# Autodesk Inventor assembly: ODrive S1 Housing Assembly
(part 2 of 2)
- C:\Users\seene\OneDrive\SBRT\Robocup Rescue\Chassis\Electronics Box\ODrive S1 Housing Assembly\C_0805_2012Metric_3.ipt
- C:\Users\seene\OneDrive\SBRT\Robocup Rescue\Chassis\Electronics Box\ODrive S1 Housing Assembly\_X2_8010632F54C130B130FC30B903A6_X0_10x9.5L_SIDE_CODE_G_3.ipt
- C:\Users\seene\OneDrive\SBRT\Robocup Rescue\Chassis\Electronics Box\ODrive S1 Housing Assembly\ASMPH-0806.ipt
- C:\Users\seene\OneDrive\SBRT\Robocup Rescue\Chassis\Electronics Box\ODrive S1 Housing Assembly\Extruded_1_1.ipt
- C:\Users\seene\OneDrive\SBRT\Robocup Rescue\Chassis\Electronics Box\ODrive S1 Housing Assembly\R_0402_1005Metric_65.ipt
- C:\Users\seene\OneDrive\SBRT\Robocup Rescue\Chassis\Electronics Box\ODrive S1 Housing Assembly\SOP_Advance(N)_(1)_11.ipt
- C:\Users\seene\OneDrive\SBRT\Robocup Rescue\Chassis\Electronics Box\ODrive S1 Housing Assembly\SOP_Advance(N)_(1)_2_4.ipt
- C:\Users\seene\OneDrive\SBRT\Robocup Rescue\Chassis\Electronics Box\ODrive S1 Housing Assembly\SOP_Advance(N)_(1)_5_4.ipt
- C:\Users\seene\OneDrive\SBRT\Robocup Rescue\Chassis\Electronics Box\ODrive S1 Housing Assembly\Open_CASCADE_STEP_translator_6.8_48.4.1_30.ipt
- C:\Users\seene\OneDrive\SBRT\Robocup Rescue\Chassis\Electronics Box\ODrive S1 Housing Assembly\Open_CASCADE_STEP_translator_6.8_48.4.1_26.ipt
- C:\Users\seene\OneDrive\SBRT\Robocup Rescue\Chassis\Electronics Box\ODrive S1 Housing Assembly\Open_CASCADE_STEP_translator_6.8_48.4.1_46.ipt
- C:\Users\seene\OneDrive\SBRT\Robocup Rescue\Chassis\Electronics Box\ODrive S1 Housing Assembly\Open_CASCADE_STEP_translator_6.8_48.4.1_42.ipt
- C:\Users\seene\OneDrive\SBRT\Robocup Rescue\Chassis\Electronics Box\ODrive S1 Housing Assembly\Open_CASCADE_STEP_translator_6.8_48.4.1_62.ipt
- C:\Users\seene\OneDrive\SBRT\Robocup Rescue\Chassis\Electronics Box\ODrive S1 Housing Assembly\Open_CASCADE_STEP_translator_6.8_48.4.1_58.ipt
- C:\Users\seene\OneDrive\SBRT\Robocup Rescue\Chassis\Electronics Box\ODrive S1 Housing Assembly\R_0402_1005Metric_25.ipt
- C:\Users\seene\OneDrive\SBRT\Robocup Rescue\Chassis\Electronics Box\ODrive S1 Housing Assembly\R_0402_1005Metric_21.ipt
- C:\Users\seene\OneDrive\SBRT\Robocup Rescue\Chassis\Electronics Box\ODrive S1 Housing Assembly\Open_CASCADE_STEP_translator_6.8_48.2.1.ipt
- C:\Users\seene\OneDrive\SBRT\Robocup Rescue\Chassis\Electronics Box\ODrive S1 Housing Assembly\Open_CASCADE_STEP_translator_6.8_56.4.1_5.ipt
- C:\Users\seene\OneDrive\SBRT\Robocup Rescue\Chassis\Electronics Box\ODrive S1 Housing Assembly\Leader_3_1.ipt
- C:\Users\seene\OneDrive\SBRT\Robocup Rescue\Chassis\Electronics Box\ODrive S1 Housing Assembly\Open_CASCADE_STEP_translator_6.8_5.2.1.ipt
- C:\Users\seene\OneDrive\SBRT\Robocup Rescue\Chassis\Electronics Box\ODrive S1 Housing Assembly\Open_CASCADE_STEP_translator_6.8_48.2.1_1.ipt
- C:\Users\seene\OneDrive\SBRT\Robocup Rescue\Chassis\Electronics Box\ODrive S1 Housing Assembly\Leader_15.ipt
- C:\Users\seene\OneDrive\SBRT\Robocup Rescue\Chassis\Electronics Box\ODrive S1 Housing Assembly\Open_CASCADE_STEP_translator_6.8_48.4.1_14.ipt
- C:\Users\seene\OneDrive\SBRT\Robocup Rescue\Chassis\Electronics Box\ODrive S1 Housing Assembly\Open_CASCADE_STEP_translator_6.8_48.4.1_10.ipt
- C:\Users\seene\OneDrive\SBRT\Robocup Rescue\Chassis\Electronics Box\ODrive S1 Housing Assembly\R_0402_1005Metric_13.ipt
- C:\Users\seene\OneDrive\SBRT\Robocup Rescue\Chassis\Electronics Box\ODrive S1 Housing Assembly\_X2_8010632F54C15EA77248752888DC52A97AEF5B5003A6_X0_10_SIZE_CODE_G_1.ipt
- C:\Users\seene\OneDrive\SBRT\Robocup Rescue\Chassis\Electronics Box\ODrive S1 Housing Assembly\C_0402_1005Metric_10.ipt
- C:\Users\seene\OneDrive\SBRT\Robocup Rescue\Chassis\Electronics Box\ODrive S1 Housing Assembly\Open_CASCADE_STEP_translator_6.8_34.4.1_7.ipt
- C:\Users\seene\OneDrive\SBRT\Robocup Rescue\Chassis\Electronics Box\ODrive S1 Housing Assembly\Open_CASCADE_STEP_translator_6.8_34.4.1_3.ipt
- C:\Users\seene\OneDrive\SBRT\Robocup Rescue\Chassis\Electronics Box\ODrive S1 Housing Assembly\Open_CASCADE_STEP_translator_6.8_41.4.1_4.ipt
- C:\Users\seene\OneDrive\SBRT\Robocup Rescue\Chassis\Electronics Box\ODrive S1 Housing Assembly\Open_CASCADE_STEP_translator_6.8_41.4.1.ipt
- C:\Users\seene\OneDrive\SBRT\Robocup Rescue\Chassis\Electronics Box\ODrive S1 Housing Assembly\Cylinder_4_1.ipt
- C:\Users\seene\OneDrive\SBRT\Robocup Rescue\Chassis\Electronics Box\ODrive S1 Housing Assembly\B0-6.3-0-2512_1.ipt
- C:\Users\seene\OneDrive\SBRT\Robocup Rescue\Chassis\Electronics Box\ODrive S1 Housing Assembly\Cylinder_17.ipt
- C:\Users\seene\OneDrive\SBRT\Robocup Rescue\Chassis\Electronics Box\ODrive S1 Housing Assembly\Cylinder_13.ipt
- C:\Users\seene\OneDrive\SBRT\Robocup Rescue\Chassis\Electronics Box\ODrive S1 Housing Assembly\Cylinder_7_1.ipt
- C:\Users\seene\OneDrive\SBRT\Robocup Rescue\Chassis\Electronics Box\ODrive S1 Housing Assembly\C_0603_1608Metric_9.ipt
- C:\Users\seene\OneDrive\SBRT\Robocup Rescue\Chassis\Electronics Box\ODrive S1 Housing Assembly\C_0603_1608Metric_5.ipt
- C:\Users\seene\OneDrive\SBRT\Robocup Rescue\Chassis\Electronics Box\ODrive S1 Housing Assembly\Pins_7.ipt
- C:\Users\seene\OneDrive\SBRT\Robocup Rescue\Chassis\Electronics Box\ODrive S1 Housing Assembly\C_0603_1608Metric.ipt
- C:\Users\seene\OneDrive\SBRT\Robocup Rescue\Chassis\Electronics Box\ODrive S1 Housing Assembly\lead_2.ipt
- C:\Users\seene\OneDrive\SBRT\Robocup Rescue\Chassis\Electronics Box\ODrive S1 Housing Assembly\Open_CASCADE_STEP_translator_6.8_2.3.1_11.ipt
- C:\Users\seene\OneDrive\SBRT\Robocup Rescue\Chassis\Electronics Box\ODrive S1 Housing Assembly\Open_CASCADE_STEP_translator_6.8_2.2.1_1.ipt
- C:\Users\seene\OneDrive\SBRT\Robocup Rescue\Chassis\Electronics Box\ODrive S1 Housing Assembly\_Dual_s.ipt
- C:\Users\seene\OneDrive\SBRT\Robocup Rescue\Chassis\Electronics Box\ODrive S1 Housing Assembly\R_0402_1005Metric_32.ipt
- C:\Users\seene\OneDrive\SBRT\Robocup Rescue\Chassis\Electronics Box\ODrive S1 Housing Assembly\R_0402_1005Metric_46.ipt
- C:\Users\seene\OneDrive\SBRT\Robocup Rescue\Chassis\Electronics Box\ODrive S1 Housing Assembly\HCS2512_L500_stp_1_2.ipt
- C:\Users\seene\OneDrive\SBRT\Robocup Rescue\Chassis\Electronics Box\ODrive S1 Housing Assembly\Open_CASCADE_STEP_translator_6.8_48.4.1_5.ipt
- C:\Users\seene\OneDrive\SBRT\Robocup Rescue\Chassis\Electronics Box\ODrive S1 Housing Assembly\Open_CASCADE_STEP_translator_6.8_48.4.1_21.ipt
- C:\Users\seene\OneDrive\SBRT\Robocup Rescue\Chassis\Electronics Box\ODrive S1 Housing Assembly\Open_CASCADE_STEP_translator_6.8_48.4.1_37.ipt
- C:\Users\seene\OneDrive\SBRT\Robocup Rescue\Chassis\Electronics Box\ODrive S1 Housing Assembly\Open_CASCADE_STEP_translator_6.8_48.4.1_53.ipt
- C:\Users\seene\OneDrive\SBRT\Robocup Rescue\Chassis\Electronics Box\ODrive S1 Housing Assembly\Leader_4_2.ipt
- C:\Users\seene\OneDrive\SBRT\Robocup Rescue\Chassis\Electronics Box\ODrive S1 Housing Assembly\Open_CASCADE_STEP_translator_6.8_56.4.1.ipt
- C:\Users\seene\OneDrive\SBRT\Robocup Rescue\Chassis\Electronics Box\ODrive S1 Housing Assembly\Leader_6_1.ipt
- C:\Users\seene\OneDrive\SBRT\Robocup Rescue\Chassis\Electronics Box\ODrive S1 Housing Assembly\Leader_10.ipt
- C:\Users\seene\OneDrive\SBRT\Robocup Rescue\Chassis\Electronics Box\ODrive S1 Housing Assembly\C_0402_1005Metric_31.ipt
- C:\Users\seene\OneDrive\SBRT\Robocup Rescue\Chassis\Electronics Box\ODrive S1 Housing Assembly\C_0805_1MM_2_1.ipt
- C:\Users\seene\OneDrive\SBRT\Robocup Rescue\Chassis\Electronics Box\ODrive S1 Housing Assembly\C_0805_1MM.ipt
- C:\Users\seene\OneDrive\SBRT\Robocup Rescue\Chassis\Electronics Box\ODrive S1 Housing Assembly\_X2_8010632F54C130EA30FC30C97DDA03A6_X0_10_SIZE_CODE_G_3.ipt
- C:\Users\seene\OneDrive\SBRT\Robocup Rescue\Chassis\Electronics Box\ODrive S1 Housing Assembly\_X2_8010632F54C15EA7724803A6_X0_10_SIZE_CODE_G_1.ipt
- C:\Users\seene\OneDrive\SBRT\Robocup Rescue\Chassis\Electronics Box\ODrive S1 Housing Assembly\R_0402_1005Metric_11.ipt
- C:\Users\seene\OneDrive\SBRT\Robocup Rescue\Chassis\Electronics Box\ODrive S1 Housing Assembly\C_0603_1608Metric_28.ipt
- C:\Users\seene\OneDrive\SBRT\Robocup Rescue\Chassis\Electronics Box\ODrive S1 Housing Assembly\_X2_8010632F54C130EA30FC30C97DDA03A6_X0_10_SIZE_CODE_G_7.ipt
- C:\Users\seene\OneDrive\SBRT\Robocup Rescue\Chassis\Electronics Box\ODrive S1 Housing Assembly\B0-6.3-0-2512_3.ipt
- C:\Users\seene\OneDrive\SBRT\Robocup Rescue\Chassis\Electronics Box\ODrive S1 Housing Assembly\C_0603_1608Metric_33.ipt
- C:\Users\seene\OneDrive\SBRT\Robocup Rescue\Chassis\Electronics Box\ODrive S1 Housing Assembly\C_0603_1608Metric_31.ipt
- C:\Users\seene\OneDrive\SBRT\Robocup Rescue\Chassis\Electronics Box\ODrive S1 Housing Assembly\Open_CASCADE_STEP_translator_6.8_34.2.1.ipt
- C:\Users\seene\OneDrive\SBRT\Robocup Rescue\Chassis\Electronics Box\ODrive S1 Housing Assembly\SOP_Advance(N)_(1)_6_3.ipt
- C:\Users\seene\OneDrive\SBRT\Robocup Rescue\Chassis\Electronics Box\ODrive S1 Housing Assembly\Open_CASCADE_STEP_translator_6.8_2.3.1_4.ipt
- C:\Users\seene\OneDrive\SBRT\Robocup Rescue\Chassis\Electronics Box\ODrive S1 Housing Assembly\_X2_00C700D000B300FD_X0_-_X2_00C000AD00C900EC_X0_2.ipt
- C:\Users\seene\OneDrive\SBRT\Robocup Rescue\Chassis\Electronics Box\ODrive S1 Housing Assembly\C_0603_1608Metric_1.ipt
- C:\Users\seene\OneDrive\SBRT\Robocup Rescue\Chassis\Electronics Box\ODrive S1 Housing Assembly\C_0402_1005Metric_13.ipt
- C:\Users\seene\OneDrive\SBRT\Robocup Rescue\Chassis\Electronics Box\ODrive S1 Housing Assembly\D_SOD-123F_5.ipt
- C:\Users\seene\OneDrive\SBRT\Robocup Rescue\Chassis\Electronics Box\ODrive S1 Housing Assembly\Cylinder_11.ipt
- C:\Users\seene\OneDrive\SBRT\Robocup Rescue\Chassis\Electronics Box\ODrive S1 Housing Assembly\M3Ò»×ÖÆ½Ô²Í·ÂÝ¶¤.ipt
- C:\Users\seene\OneDrive\SBRT\Robocup Rescue\Chassis\Electronics Box\ODrive S1 Housing Assembly\C_0402_1005Metric_23.ipt
- C:\Users\seene\OneDrive\SBRT\Robocup Rescue\Chassis\Electronics Box\ODrive S1 Housing Assembly\C_0402_1005Metric_19.ipt
- C:\Users\seene\OneDrive\SBRT\Robocup Rescue\Chassis\Electronics Box\ODrive S1 Housing Assembly\Cylinder_24.ipt
- C:\Users\seene\OneDrive\SBRT\Robocup Rescue\Chassis\Electronics Box\ODrive S1 Housing Assembly\R_0402_1005Metric_5.ipt
- C:\Users\seene\OneDrive\SBRT\Robocup Rescue\Chassis\Electronics Box\ODrive S1 Housing Assembly\SOP_Advance(N)_(1)_1_4.ipt
- C:\Users\seene\OneDrive\SBRT\Robocup Rescue\Chassis\Electronics Box\ODrive S1 Housing Assembly\SOP_Advance(N)_(1)_12.ipt
- C:\Users\seene\OneDrive\SBRT\Robocup Rescue\Chassis\Electronics Box\ODrive S1 Housing Assembly\SOP_Advance(N)_(1)_4_4.ipt
- C:\Users\seene\OneDrive\SBRT\Robocup Rescue\Chassis\Electronics Box\ODrive S1 Housing Assembly\SOP_Advance(N)_(1)_3_5.ipt
- C:\Users\seene\OneDrive\SBRT\Robocup Rescue\Chassis\Electronics Box\ODrive S1 Housing Assembly\SOP_Advance(N)_(1)_6_4.ipt
- C:\Users\seene\OneDrive\SBRT\Robocup Rescue\Chassis\Electronics Box\ODrive S1 Housing Assembly\R_0402_1005Metric_41.ipt
- C:\Users\seene\OneDrive\SBRT\Robocup Rescue\Chassis\Electronics Box\ODrive S1 Housing Assembly\R_0402_1005Metric_37.ipt
- C:\Users\seene\OneDrive\SBRT\Robocup Rescue\Chassis\Electronics Box\ODrive S1 Housing Assembly\R_0603_1608Metric_2.ipt
- C:\Users\seene\OneDrive\SBRT\Robocup Rescue\Chassis\Electronics Box\ODrive S1 Housing Assembly\R_0402_1005Metric_48.ipt
- C:\Users\seene\OneDrive\SBRT\Robocup Rescue\Chassis\Electronics Box\ODrive S1 Housing Assembly\R_0402_1005Metric_58.ipt
- C:\Users\seene\OneDrive\SBRT\Robocup Rescue\Chassis\Electronics Box\ODrive S1 Housing Assembly\HCS2512_L500_stp_3_2.ipt
- C:\Users\seene\OneDrive\SBRT\Robocup Rescue\Chassis\Electronics Box\ODrive S1 Housing Assembly\R_0402_1005Metric_70.ipt
- C:\Users\seene\OneDrive\SBRT\Robocup Rescue\Chassis\Electronics Box\ODrive S1 Housing Assembly\R_0402_1005Metric_66.ipt
- C:\Users\seene\OneDrive\SBRT\Robocup Rescue\Chassis\Electronics Box\ODrive S1 Housing Assembly\C_0805_1MM_5_1.ipt
- C:\Users\seene\OneDrive\SBRT\Robocup Rescue\Chassis\Electronics Box\ODrive S1 Housing Assembly\C_0402_1005Metric_44.ipt
- C:\Users\seene\OneDrive\SBRT\Robocup Rescue\Chassis\Electronics Box\ODrive S1 Housing Assembly\C_0603_1608Metric_18.ipt
- C:\Users\seene\OneDrive\SBRT\Robocup Rescue\Chassis\Electronics Box\ODrive S1 Housing Assembly\C_0805_2012Metric.ipt
- C:\Users\seene\OneDrive\SBRT\Robocup Rescue\Chassis\Electronics Box\ODrive S1 Housing Assembly\C_0805_2012Metric_2.ipt
- C:\Users\seene\OneDrive\SBRT\Robocup Rescue\Chassis\Electronics Box\ODrive S1 Housing Assembly\_X2_8010632F54C130EA30FC30C97DDA03A6_X0_10_SIZE_CODE_G_5.ipt
- C:\Users\seene\OneDrive\SBRT\Robocup Rescue\Chassis\Electronics Box\ODrive S1 Housing Assembly\SOP_Advance(N)_(1)_7_5.ipt
- C:\Users\seene\OneDrive\SBRT\Robocup Rescue\Chassis\Electronics Box\ODrive S1 Housing Assembly\Extruded_11.ipt
- C:\Users\seene\OneDrive\SBRT\Robocup Rescue\Chassis\Electronics Box\ODrive S1 Housing Assembly\R_0402_1005Metric_64.ipt
- C:\Users\seene\OneDrive\SBRT\Robocup Rescue\Chassis\Electronics Box\ODrive S1 Housing Assembly\SOT23-3_1.ipt
- C:\Users\seene\OneDrive\SBRT\Robocup Rescue\Chassis\Electronics Box\ODrive S1 Housing Assembly\SOP_Advance(N)_(1)_2_5.ipt
- C:\Users\seene\OneDrive\SBRT\Robocup Rescue\Chassis\Electronics Box\ODrive S1 Housing Assembly\SOP_Advance(N)_(1)_5_5.ipt
- C:\Users\seene\OneDrive\SBRT\Robocup Rescue\Chassis\Electronics Box\ODrive S1 Housing Assembly\_CAS_c_D2A.ipt
- C:\Users\seene\OneDrive\SBRT\Robocup Rescue\Chassis\Electronics Box\ODrive S1 Housing Assembly\R_0402_1005Metric_31.ipt
- C:\Users\seene\OneDrive\SBRT\Robocup Rescue\Chassis\Electronics Box\ODrive S1 Housing Assembly\R_0402_1005Metric_45.ipt
- C:\Users\seene\OneDrive\SBRT\Robocup Rescue\Chassis\Electronics Box\ODrive S1 Housing Assembly\HCS2512_L500_stp_1_3.ipt
- C:\Users\seene\OneDrive\SBRT\Robocup Rescue\Chassis\Electronics Box\ODrive S1 Housing Assembly\Leader_2_2.ipt
- C:\Users\seene\OneDrive\SBRT\Robocup Rescue\Chassis\Electronics Box\ODrive S1 Housing Assembly\Open_CASCADE_STEP_translator_6.8_48.4.1_13.ipt
- C:\Users\seene\OneDrive\SBRT\Robocup Rescue\Chassis\Electronics Box\ODrive S1 Housing Assembly\BM05B-GHS-TBT.ipt
- C:\Users\seene\OneDrive\SBRT\Robocup Rescue\Chassis\Electronics Box\ODrive S1 Housing Assembly\_X2_8010632F54C15EA77248752888DC52A97AEF5B5003A6_X0_10_SIZE_CODE_G.ipt
- C:\Users\seene\OneDrive\SBRT\Robocup Rescue\Chassis\Electronics Box\ODrive S1 Housing Assembly\Open_CASCADE_STEP_translator_6.8_34.4.1_6.ipt
- C:\Users\seene\OneDrive\SBRT\Robocup Rescue\Chassis\Electronics Box\ODrive S1 Housing Assembly\Open_CASCADE_STEP_translator_6.8_41.4.1_3.ipt
- C:\Users\seene\OneDrive\SBRT\Robocup Rescue\Chassis\Electronics Box\ODrive S1 Housing Assembly\Cylinder_3_2.ipt
- C:\Users\seene\OneDrive\SBRT\Robocup Rescue\Chassis\Electronics Box\ODrive S1 Housing Assembly\Cylinder_16.ipt
- C:\Users\seene\OneDrive\SBRT\Robocup Rescue\Chassis\Electronics Box\ODrive S1 Housing Assembly\R_0402_1005Metric_7.ipt
- C:\Users\seene\OneDrive\SBRT\Robocup Rescue\Chassis\Electronics Box\ODrive S1 Housing Assembly\C_0603_1608Metric_8.ipt
- C:\Users\seene\OneDrive\SBRT\Robocup Rescue\Chassis\Electronics Box\ODrive S1 Housing Assembly\Pins_8.ipt
- C:\Users\seene\OneDrive\SBRT\Robocup Rescue\Chassis\Electronics Box\ODrive S1 Housing Assembly\C_0402_1005Metric_4.ipt
- C:\Users\seene\OneDrive\SBRT\Robocup Rescue\Chassis\Electronics Box\ODrive S1 Housing Assembly\Open_CASCADE_STEP_translator_6.8_2.3.1_10.ipt
- C:\Users\seene\OneDrive\SBRT\Robocup Rescue\Chassis\Electronics Box\ODrive S1 Housing Assembly\Open_CASCADE_STEP_translator_6.8_48.4.1_4.ipt
- C:\Users\seene\OneDrive\SBRT\Robocup Rescue\Chassis\Electronics Box\ODrive S1 Housing Assembly\Open_CASCADE_STEP_translator_6.8_48.4.1_20.ipt
- C:\Users\seene\OneDrive\SBRT\Robocup Rescue\Chassis\Electronics Box\ODrive S1 Housing Assembly\Open_CASCADE_STEP_translator_6.8_48.4.1_36.ipt
- C:\Users\seene\OneDrive\SBRT\Robocup Rescue\Chassis\Electronics Box\ODrive S1 Housing Assembly\Open_CASCADE_STEP_translator_6.8_48.4.1_52.ipt
- C:\Users\seene\OneDrive\SBRT\Robocup Rescue\Chassis\Electronics Box\ODrive S1 Housing Assembly\Leader_3_2.ipt
- C:\Users\seene\OneDrive\SBRT\Robocup Rescue\Chassis\Electronics Box\ODrive S1 Housing Assembly\Thermal_Shape_3.ipt
- C:\Users\seene\OneDrive\SBRT\Robocup Rescue\Chassis\Electronics Box\ODrive S1 Housing Assembly\Leader_5_3.ipt
- C:\Users\seene\OneDrive\SBRT\Robocup Rescue\Chassis\Electronics Box\ODrive S1 Housing Assembly\Leader_9_1.ipt
- C:\Users\seene\OneDrive\SBRT\Robocup Rescue\Chassis\Electronics Box\ODrive S1 Housing Assembly\C_0603_1608Metric_25.ipt
- C:\Users\seene\OneDrive\SBRT\Robocup Rescue\Chassis\Electronics Box\ODrive S1 Housing Assembly\C_0805_1MM_6.ipt
- C:\Users\seene\OneDrive\SBRT\Robocup Rescue\Chassis\Electronics Box\ODrive S1 Housing Assembly\_X2_8010632F54C130EA30FC30C97DDA03A6_X0_10_SIZE_CODE_G_2.ipt
- C:\Users\seene\OneDrive\SBRT\Robocup Rescue\Chassis\Electronics Box\ODrive S1 Housing Assembly\RES_0603_(1608_metric).ipt
- C:\Users\seene\OneDrive\SBRT\Robocup Rescue\Chassis\Electronics Box\ODrive S1 Housing Assembly\C_0603_1608Metric_27.ipt
- C:\Users\seene\OneDrive\SBRT\Robocup Rescue\Chassis\Electronics Box\ODrive S1 Housing Assembly\C_0402_1005Metric_9.ipt
- C:\Users\seene\OneDrive\SBRT\Robocup Rescue\Chassis\Electronics Box\ODrive S1 Housing Assembly\C_0402_1005Metric_41.ipt
- C:\Users\seene\OneDrive\SBRT\Robocup Rescue\Chassis\Electronics Box\ODrive S1 Housing Assembly\SOP_Advance(N)_(1)_6_5.ipt
- C:\Users\seene\OneDrive\SBRT\Robocup Rescue\Chassis\Electronics Box\ODrive S1 Housing Assembly\Open_CASCADE_STEP_translator_6.8_2.3.1_3.ipt
- C:\Users\seene\OneDrive\SBRT\Robocup Rescue\Chassis\Electronics Box\ODrive S1 Housing Assembly\NONE.ipt
- C:\Users\seene\OneDrive\SBRT\Robocup Rescue\Chassis\Electronics Box\ODrive S1 Housing Assembly\C_0402_1005Metric_6.ipt
- C:\Users\seene\OneDrive\SBRT\Robocup Rescue\Chassis\Electronics Box\ODrive S1 Housing Assembly\C_0402_1005Metric_12.ipt
- C:\Users\seene\OneDrive\SBRT\Robocup Rescue\Chassis\Electronics Box\ODrive S1 Housing Assembly\Cylinder_10.ipt
- C:\Users\seene\OneDrive\SBRT\Robocup Rescue\Chassis\Electronics Box\ODrive S1 Housing Assembly\º¸½Å_1.ipt
- C:\Users\seene\OneDrive\SBRT\Robocup Rescue\Chassis\Electronics Box\ODrive S1 Housing Assembly\C_0402_1005Metric_22.ipt
- C:\Users\seene\OneDrive\SBRT\Robocup Rescue\Chassis\Electronics Box\ODrive S1 Housing Assembly\Cylinder_23.ipt
- C:\Users\seene\OneDrive\SBRT\Robocup Rescue\Chassis\Electronics Box\ODrive S1 Housing Assembly\Extruded_12.ipt
- C:\Users\seene\OneDrive\SBRT\Robocup Rescue\Chassis\Electronics Box\ODrive S1 Housing Assembly\SOP_Advance(N)_(1)_1_5.ipt
- C:\Users\seene\OneDrive\SBRT\Robocup Rescue\Chassis\Electronics Box\ODrive S1 Housing Assembly\SOP_Advance(N)_(1)_4_5.ipt
- C:\Users\seene\OneDrive\SBRT\Robocup Rescue\Chassis\Electronics Box\ODrive S1 Housing Assembly\R_0402_1005Metric_40.ipt
- C:\Users\seene\OneDrive\SBRT\Robocup Rescue\Chassis\Electronics Box\ODrive S1 Housing Assembly\R_0402_1005Metric_51.ipt
- C:\Users\seene\OneDrive\SBRT\Robocup Rescue\Chassis\Electronics Box\ODrive S1 Housing Assembly\R_0402_1005Metric_57.ipt
- C:\Users\seene\OneDrive\SBRT\Robocup Rescue\Chassis\Electronics Box\ODrive S1 Housing Assembly\R_0402_1005Metric_69.ipt
- C:\Users\seene\OneDrive\SBRT\Robocup Rescue\Chassis\Electronics Box\ODrive S1 Housing Assembly\Open_CASCADE_STEP_translator_6.8_48.4.1_29.ipt
- C:\Users\seene\OneDrive\SBRT\Robocup Rescue\Chassis\Electronics Box\ODrive S1 Housing Assembly\Open_CASCADE_STEP_translator_6.8_48.4.1_45.ipt
- C:\Users\seene\OneDrive\SBRT\Robocup Rescue\Chassis\Electronics Box\ODrive S1 Housing Assembly\Open_CASCADE_STEP_translator_6.8_48.4.1_61.ipt
- C:\Users\seene\OneDrive\SBRT\Robocup Rescue\Chassis\Electronics Box\ODrive S1 Housing Assembly\R_0402_1005Metric_24.ipt
## Components (552 placed, 552 different names)
1. NAUO1
2. NAUO2
3. NAUO3
4. NAUO4
5. NAUO5
6. NAUO6
7. NAUO7
8. NAUO8
9. NAUO9
10. NAUO10
11. NAUO11
12. NAUO12
13. NAUO13
14. NAUO14
15. NAUO15
16. NAUO16
17. NAUO17
18. NAUO18
19. NAUO19
20. NAUO20
21. NAUO21
22. NAUO22
23. NAUO23
24. NAUO24
25. NAUO25
26. NAUO26
27. NAUO27
28. NAUO28
29. NAUO29
30. NAUO30
31. NAUO31
32. NAUO32
33. NAUO33
34. NAUO34
35. NAUO35
36. NAUO36
37. NAUO37
38. NAUO38
39. NAUO39
40. NAUO40
41. NAUO41
42. NAUO42
43. NAUO43
44. NAUO44
45. NAUO45
46. NAUO46
47. NAUO47
48. NAUO48
49. NAUO49
50. NAUO50
51. NAUO51
52. NAUO52
53. NAUO53
54. NAUO54
55. NAUO55
56. NAUO56
57. NAUO57
58. NAUO58
59. NAUO59
60. NAUO60
61. NAUO61
62. NAUO62
63. NAUO63
64. NAUO64
65. NAUO65
66. NAUO66
67. NAUO67
68. NAUO68
69. NAUO69
70. NAUO70
71. NAUO71
72. NAUO72
73. NAUO73
74. NAUO74
75. NAUO75
76. NAUO76
77. NAUO77
78. NAUO78
79. NAUO79
80. NAUO80
81. NAUO81
82. NAUO82
83. NAUO83
84. NAUO84
85. NAUO85
86. NAUO86
87. NAUO87
88. NAUO88
89. NAUO89
90. NAUO90
91. NAUO91
92. NAUO92
93. NAUO93
94. NAUO94
95. NAUO95
96. NAUO96
97. NAUO97
98. NAUO98
99. NAUO99
100. NAUO100
101. NAUO101
102. NAUO102
103. NAUO103
104. NAUO104
105. NAUO105
106. NAUO106
107. NAUO107
108. NAUO108
109. NAUO109
110. NAUO110
111. NAUO111
112. NAUO112
113. NAUO113
114. NAUO114
115. NAUO115
116. NAUO116
117. NAUO117
118. NAUO118
119. NAUO119
120. NAUO120
121. NAUO121
122. NAUO122
123. NAUO123
124. NAUO124
125. NAUO125
126. NAUO126
127. NAUO127
128. NAUO128
129. NAUO129
130. NAUO130
131. NAUO131
132. NAUO132
133. NAUO133
134. NAUO134
135. NAUO135
136. NAUO136
137. NAUO137
138. NAUO138
139. NAUO139
140. NAUO140
141. NAUO141
142. NAUO142
143. NAUO143
144. NAUO144
145. NAUO145
146. NAUO146
147. NAUO147
148. NAUO148
149. NAUO149
150. NAUO150
151. NAUO151
152. NAUO152
153. NAUO153
154. NAUO154
155. NAUO155
156. NAUO156
157. NAUO157
158. NAUO158
159. NAUO159
160. NAUO160
161. NAUO161
162. NAUO162
163. NAUO163
164. NAUO164
165. NAUO165
166. NAUO166
167. NAUO167
168. NAUO168
169. NAUO169
170. NAUO170
171. NAUO171
172. NAUO172
173. NAUO173
174. NAUO174
175. NAUO175
176. NAUO176
177. NAUO177
178. NAUO178
179. NAUO179
180. NAUO180
181. NAUO181
182. NAUO182
183. NAUO183
184. NAUO184
185. NAUO185
186. NAUO186
187. NAUO187
188. NAUO188
189. NAUO189
190. NAUO190
191. NAUO191
192. NAUO192
193. NAUO193
194. NAUO194
195. NAUO195
196. NAUO196
197. NAUO197
198. NAUO198
199. NAUO199
200. NAUO200
201. NAUO201
202. NAUO202
203. NAUO203
204. NAUO204
205. NAUO205
206. NAUO206
207. NAUO207
208. NAUO208
209. NAUO209
210. NAUO210
211. NAUO211
212. NAUO212
213. NAUO213
214. NAUO214
215. NAUO215
216. NAUO216
217. NAUO217
218. NAUO218
219. NAUO219
220. NAUO220
221. NAUO221
222. NAUO222
223. NAUO223
224. NAUO224
225. NAUO225
226. NAUO226
227. NAUO227
228. NAUO228
229. NAUO229
230. NAUO230
231. NAUO231
232. NAUO232
233. NAUO233
234. NAUO234
235. NAUO235
236. NAUO236
237. NAUO237
238. NAUO238
239. NAUO239
240. NAUO240
241. NAUO241
242. NAUO242
243. NAUO243
244. NAUO244
245. NAUO245
246. NAUO246
247. NAUO247
248. NAUO248
249. NAUO249
250. NAUO250
251. NAUO251
252. NAUO252
253. NAUO253
254. NAUO254
255. NAUO255
256. NAUO256
257. NAUO257
258. NAUO258
259. NAUO259
260. NAUO260
261. NAUO261
262. NAUO262
263. NAUO263
264. NAUO264
265. NAUO265
266. NAUO266
267. NAUO267
268. NAUO268
269. NAUO269
270. NAUO270
271. NAUO271
272. NAUO272
273. NAUO273
274. NAUO274
275. NAUO275
276. NAUO276
277. NAUO277
278. NAUO278
279. NAUO279
280. NAUO280
281. NAUO281
282. NAUO282
283. NAUO283
284. NAUO284
285. NAUO285
286. NAUO286
287. NAUO287
288. NAUO288
289. NAUO289
290. NAUO290
291. NAUO291
292. NAUO292
293. NAUO293
294. NAUO294
295. NAUO295
296. NAUO296
297. NAUO297
298. NAUO298
299. NAUO299
300. NAUO300
301. NAUO301
302. NAUO302
303. NAUO303
304. NAUO304
305. NAUO305
306. NAUO306
307. NAUO307
308. NAUO308
309. NAUO309
310. NAUO310
311. NAUO311
312. NAUO312
313. NAUO313
314. NAUO314
315. NAUO315
316. NAUO316
317. NAUO317
318. NAUO318
319. NAUO319
320. NAUO320
321. NAUO321
322. NAUO322
323. NAUO323
324. NAUO324
325. NAUO325
326. NAUO326
327. NAUO327
328. NAUO328
329. NAUO329
330. NAUO330
331. NAUO331
332. NAUO332
333. NAUO333
334. NAUO334
335. NAUO335
336. NAUO336
337. NAUO337
338. NAUO338
339. NAUO339
340. NAUO340
341. NAUO341
342. NAUO342
343. NAUO343
344. NAUO344
345. NAUO345
346. NAUO346
347. NAUO347
348. NAUO348
349. NAUO349
350. NAUO350
351. NAUO351
352. NAUO352
353. NAUO353
354. NAUO354
355. NAUO355
356. NAUO356
357. NAUO357
358. NAUO358
359. NAUO359
360. NAUO360
361. NAUO361
362. NAUO362
363. NAUO363
364. NAUO364
365. NAUO365
366. NAUO366
367. NAUO367
368. NAUO368
369. NAUO369
370. NAUO370
371. NAUO371
372. NAUO372
373. NAUO373
374. NAUO374
375. NAUO375
376. NAUO376
377. NAUO377
378. NAUO378
379. NAUO379
380. NAUO380
381. NAUO381
382. NAUO382
383. NAUO383
384. NAUO384
385. NAUO385
386. NAUO386
387. NAUO387
388. NAUO388
389. NAUO389
390. NAUO390
391. NAUO391
392. NAUO392
393. NAUO393
394. NAUO394
395. NAUO395
396. NAUO396
397. NAUO397
398. NAUO398
399. NAUO399
400. NAUO400
401. NAUO401
402. NAUO402
403. NAUO403
404. NAUO404
405. NAUO405
406. NAUO406
407. NAUO407
408. NAUO408
409. NAUO409
410. NAUO410
411. NAUO411
412. NAUO412
413. NAUO413
414. NAUO414
415. NAUO415
416. NAUO416
417. NAUO417
418. NAUO418
419. NAUO419
420. NAUO420
421. NAUO421
422. NAUO422
423. NAUO423
424. NAUO424
425. NAUO425
426. NAUO426
427. NAUO427
428. NAUO428
429. NAUO429
430. NAUO430
431. NAUO431
432. NAUO432
433. NAUO433
434. NAUO434
435. NAUO435
436. NAUO436
437. NAUO437
438. NAUO438
439. NAUO439
440. NAUO440
441. NAUO441
442. NAUO442
443. NAUO443
444. NAUO444
445. NAUO445
446. NAUO446
447. NAUO447
448. NAUO448
449. NAUO449
450. NAUO450
451. NAUO451
452. NAUO452
453. NAUO453
454. NAUO454
455. NAUO455
456. NAUO456
457. NAUO457
458. NAUO458
459. NAUO459
460. NAUO460
461. NAUO461
462. NAUO462
463. NAUO463
464. NAUO464
465. NAUO465
466. NAUO466
467. NAUO467
468. NAUO468
469. NAUO469
470. NAUO470
471. NAUO471
472. NAUO472
473. NAUO473
474. NAUO474
475. NAUO475
476. NAUO476
477. NAUO477
478. NAUO478
479. NAUO479
480. NAUO480
481. NAUO481
482. NAUO482
483. NAUO483
484. NAUO484
485. NAUO485
486. NAUO486
487. NAUO487
488. NAUO488
489. NAUO489
490. NAUO490
491. NAUO491
492. NAUO492
493. NAUO493
494. NAUO494
495. NAUO495
496. NAUO496
497. NAUO497
498. NAUO498
499. NAUO499
500. NAUO500
501. NAUO501
502. NAUO502
503. NAUO503
504. NAUO504
505. NAUO505
506. NAUO506
507. NAUO507
508. NAUO508
509. NAUO509
510. NAUO510
511. NAUO511
512. NAUO512
513. NAUO513
514. NAUO514
515. NAUO515
516. NAUO516
517. NAUO517
518. NAUO518
519. NAUO519
520. NAUO520
521. NAUO521
522. NAUO522
523. NAUO523
524. NAUO524
525. NAUO525
526. NAUO526
527. NAUO527
528. NAUO528
529. NAUO529
530. NAUO530
531. NAUO531
532. NAUO532
533. NAUO533
534. NAUO534
535. NAUO535
536. NAUO536
537. NAUO537
538. NAUO538
539. NAUO539
540. NAUO540
541. NAUO541
542. NAUO542
543. NAUO543
544. NAUO544
545. NAUO545
546. NAUO546
547. NAUO547
548. NAUO548
549. NAUO549
550. NAUO550
551. NAUO551
552. NAUO552
